# Autodesk Inventor assembly: Another
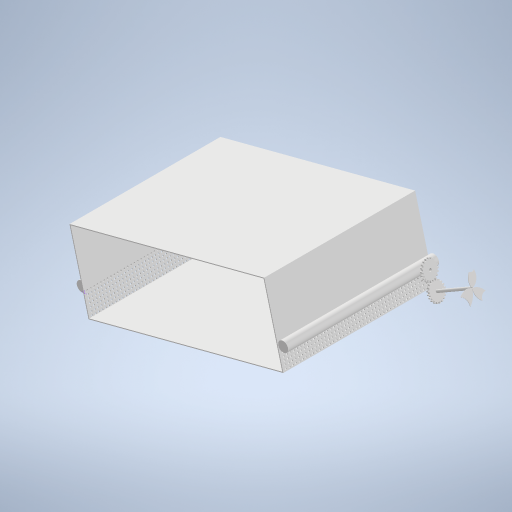
[picture p0: Inventor's stored thumbnail of the model, 512x512]
Saved by Autodesk Inventor 2024 (Build 280153000, 153)
## iProperties
Created: 2024-09-09
Part Number: Another
Document SubType Name: Assembly
Designer: srira
Author: srira
## Documents named in this file (7)
- C:\Users\srira\Documents\IITGN\3rd year\Sem5\ES408\Tentative Model\Another.iam
- C:\Users\srira\Documents\IITGN\3rd year\Sem5\ES408\Tentative Model\Dustbin Body.ipt
- C:\Users\srira\Documents\IITGN\3rd year\Sem5\ES408\Tentative Model\PVC.ipt
- C:\Users\srira\Documents\IITGN\3rd year\Sem5\ES408\Tentative Model\ranpro.ipt
- C:\Users\srira\Documents\IITGN\3rd year\Sem5\ES408\Tentative Model\Ger.ipt
- C:\Users\srira\Documents\IITGN\3rd year\Sem5\ES408\Tentative Model\ranpro_MIR.ipt
- C:\Users\srira\Documents\IITGN\3rd year\Sem5\ES408\Tentative Model\Ger_MIR.ipt
## Components (9 placed, 6 different names)
1. Dustbin Body:1 — Tangent:1, Tangent:2
2. PVC:1 — Tangent:1
3. PVC:2 — Tangent:2
4. ranpro:2 — Insert:1
5. Ger:1 — Mate:3
6. Ger:2 — Insert:1, Mate:3
7. ranpro_MIR:1 — Insert:2
8. Ger_MIR:1 — Mate:4
9. Ger_MIR:2 — Mate:4, Insert:2
## Relationships (6: Tangent 2, Insert 2, Mate 2)
- Tangent:1: Dustbin Body:1 ↔ PVC:1
- Tangent:2: Dustbin Body:1 ↔ PVC:2
- Insert:1: ranpro:2 ↔ Ger:2
- Mate:3: Ger:1 ↔ Ger:2
- Mate:4: Ger_MIR:1 ↔ Ger_MIR:2
- Insert:2: ranpro_MIR:1 ↔ Ger_MIR:2
